# Autodesk Inventor assembly: 외곽프레임
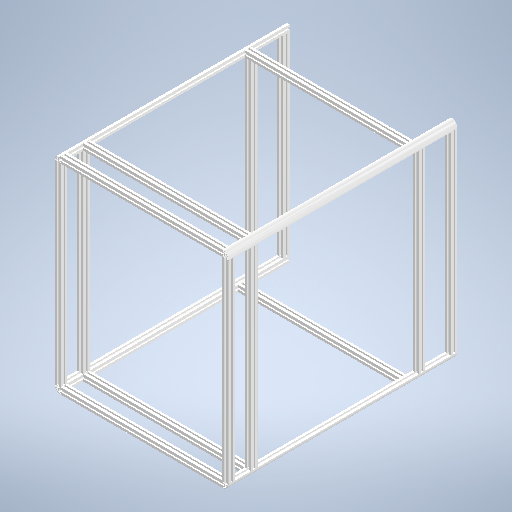
[picture p0: Inventor's stored thumbnail of the model, 512x512]
Saved by Autodesk Inventor 2025.4 (Build 294407000, 407)
## iProperties
Created: 2026-06-05
Part Number: 외곽프레임
Document SubType Name: Assembly
Designer: dalbi
Author: dalbi
## Documents named in this file (4)
- C:\Users\dalbi\OneDrive\바탕 화면\트리보 설계파일\최종 설계 파일(조립시 참고할 파일)\외곽프레임.iam
- C:\Users\dalbi\OneDrive\바탕 화면\트리보 설계파일\최종 설계 파일(조립시 참고할 파일)\AL_Profile_Round_20X20_710.ipt
- C:\Users\dalbi\OneDrive\바탕 화면\트리보 설계파일\최종 설계 파일(조립시 참고할 파일)\AL_Profile_20X20_600.ipt
- C:\Users\dalbi\OneDrive\바탕 화면\트리보 설계파일\최종 설계 파일(조립시 참고할 파일)\AL_Profile_20X20_500.ipt
## Components (18 placed, 3 different names)
1. AL_Profile_Round_20X20_710:1 — 플러쉬:1, 메이트:1, 각도:1, 메이트:2, 각도:2, 플러쉬:2, 플러쉬:7, 메이트:24, 플러쉬:24, 플러쉬:25, 메이트:25, 메이트:30, 플러쉬:34
2. AL_Profile_Round_20X20_710:2 — 플러쉬:1, 메이트:1, 각도:1, 플러쉬:4, 플러쉬:6, 플러쉬:7, 메이트:5, 플러쉬:10, 플러쉬:14, 메이트:10, 플러쉬:15, 플러쉬:26
3. AL_Profile_Round_20X20_710:3 — 각도:3, 메이트:3, 플러쉬:3, 플러쉬:4, 플러쉬:5, 플러쉬:6, 메이트:4, 플러쉬:8, 플러쉬:9, 플러쉬:16, 메이트:18, 플러쉬:23
4. AL_Profile_Round_20X20_710:4 — 메이트:2, 각도:2, 각도:3, 메이트:3, 플러쉬:2, 플러쉬:3, 플러쉬:5, 플러쉬:11, 메이트:6, 플러쉬:12, 플러쉬:13, 메이트:7, 플러쉬:17, 메이트:19, 플러쉬:18, 메이트:20, 플러쉬:19, 플러쉬:21, 메이트:26, 플러쉬:28, 메이트:27, 플러쉬:30
5. AL_Profile_20X20_600:1 — 메이트:4, 플러쉬:8, 플러쉬:9, 메이트:28
6. AL_Profile_20X20_600:2 — 플러쉬:11, 메이트:6, 플러쉬:12, 메이트:8
7. AL_Profile_20X20_600:3 — 메이트:17, 플러쉬:16, 메이트:18, 플러쉬:27
8. AL_Profile_20X20_600:4 — 메이트:5, 플러쉬:10, 메이트:28, 메이트:31
9. AL_Profile_20X20_600:5 — 플러쉬:14, 메이트:10, 플러쉬:15, 메이트:17
10. AL_Profile_20X20_600:6 — 플러쉬:13, 메이트:7, 메이트:8, 메이트:22, 플러쉬:35
11. AL_Profile_20X20_600:7 — 플러쉬:17, 메이트:19, 플러쉬:18, 메이트:21
12. AL_Profile_20X20_600:8 — 메이트:20, 플러쉬:19, 메이트:21, 플러쉬:29
13. AL_Profile_20X20_500:1 — 메이트:22, 플러쉬:21, 플러쉬:23
14. AL_Profile_20X20_500:3 — 메이트:26, 플러쉬:28, 플러쉬:29
15. AL_Profile_20X20_500:4 — 메이트:27, 플러쉬:30, 메이트:31
16. AL_Profile_20X20_500:5 — 메이트:24, 플러쉬:24, 플러쉬:25
17. AL_Profile_20X20_500:6 — 메이트:25, 플러쉬:26, 플러쉬:27
18. AL_Profile_20X20_500:8 — 메이트:30, 플러쉬:34, 플러쉬:35
## Relationships (55: Flush 30, Mate 22, Angle 3)
- 플러쉬:1 [Flush]: AL_Profile_Round_20X20_710:1 ↔ AL_Profile_Round_20X20_710:2
- 메이트:1 [Mate] (500 mm): AL_Profile_Round_20X20_710:1 ↔ AL_Profile_Round_20X20_710:2
- 각도:1 [Angle] (0 deg): AL_Profile_Round_20X20_710:1 ↔ AL_Profile_Round_20X20_710:2
- 메이트:2 [Mate] (600 mm): AL_Profile_Round_20X20_710:1 ↔ AL_Profile_Round_20X20_710:4
- 각도:2 [Angle] (0 deg): AL_Profile_Round_20X20_710:1 ↔ AL_Profile_Round_20X20_710:4
- 각도:3 [Angle] (0 deg): AL_Profile_Round_20X20_710:3 ↔ AL_Profile_Round_20X20_710:4
- 메이트:3 [Mate] (500 mm): AL_Profile_Round_20X20_710:3 ↔ AL_Profile_Round_20X20_710:4
- 플러쉬:2 [Flush]: AL_Profile_Round_20X20_710:1 ↔ AL_Profile_Round_20X20_710:4
- 플러쉬:3 [Flush]: AL_Profile_Round_20X20_710:3 ↔ AL_Profile_Round_20X20_710:4
- 플러쉬:4 [Flush]: AL_Profile_Round_20X20_710:2 ↔ AL_Profile_Round_20X20_710:3
- 플러쉬:5 [Flush]: AL_Profile_Round_20X20_710:3 ↔ AL_Profile_Round_20X20_710:4
- 플러쉬:6 [Flush]: AL_Profile_Round_20X20_710:2 ↔ AL_Profile_Round_20X20_710:3
- 플러쉬:7 [Flush]: AL_Profile_Round_20X20_710:1 ↔ AL_Profile_Round_20X20_710:2
- 메이트:4 [Mate]: AL_Profile_Round_20X20_710:3 ↔ AL_Profile_20X20_600:1
- 플러쉬:8 [Flush]: AL_Profile_Round_20X20_710:3 ↔ AL_Profile_20X20_600:1
- 플러쉬:9 [Flush]: AL_Profile_Round_20X20_710:3 ↔ AL_Profile_20X20_600:1
- 메이트:5 [Mate]: AL_Profile_Round_20X20_710:2 ↔ AL_Profile_20X20_600:4
- 플러쉬:10 [Flush]: AL_Profile_Round_20X20_710:2 ↔ AL_Profile_20X20_600:4
- 플러쉬:11 [Flush]: AL_Profile_Round_20X20_710:4 ↔ AL_Profile_20X20_600:2
- 메이트:6 [Mate]: AL_Profile_Round_20X20_710:4 ↔ AL_Profile_20X20_600:2
- 플러쉬:12 [Flush]: AL_Profile_Round_20X20_710:4 ↔ AL_Profile_20X20_600:2
- 플러쉬:13 [Flush]: AL_Profile_Round_20X20_710:4 ↔ AL_Profile_20X20_600:6
- 메이트:7 [Mate]: AL_Profile_Round_20X20_710:4 ↔ AL_Profile_20X20_600:6
- 메이트:8 [Mate] (80 mm): AL_Profile_20X20_600:2 ↔ AL_Profile_20X20_600:6
- 플러쉬:14 [Flush]: AL_Profile_Round_20X20_710:2 ↔ AL_Profile_20X20_600:5
- 메이트:10 [Mate]: AL_Profile_Round_20X20_710:2 ↔ AL_Profile_20X20_600:5
- 플러쉬:15 [Flush]: AL_Profile_Round_20X20_710:2 ↔ AL_Profile_20X20_600:5
- 메이트:17 [Mate] (50 mm): AL_Profile_20X20_600:3 ↔ AL_Profile_20X20_600:5
- 플러쉬:16 [Flush]: AL_Profile_Round_20X20_710:3 ↔ AL_Profile_20X20_600:3
- 메이트:18 [Mate]: AL_Profile_Round_20X20_710:3 ↔ AL_Profile_20X20_600:3
- 플러쉬:17 [Flush]: AL_Profile_Round_20X20_710:4 ↔ AL_Profile_20X20_600:7
- 메이트:19 [Mate]: AL_Profile_Round_20X20_710:4 ↔ AL_Profile_20X20_600:7
- 플러쉬:18 [Flush]: AL_Profile_Round_20X20_710:4 ↔ AL_Profile_20X20_600:7
- 메이트:20 [Mate]: AL_Profile_Round_20X20_710:4 ↔ AL_Profile_20X20_600:8
- 플러쉬:19 [Flush]: AL_Profile_Round_20X20_710:4 ↔ AL_Profile_20X20_600:8
- 메이트:21 [Mate] (50 mm): AL_Profile_20X20_600:7 ↔ AL_Profile_20X20_600:8
- 메이트:22 [Mate]: AL_Profile_20X20_600:6 ↔ AL_Profile_20X20_500:1
- 플러쉬:21 [Flush]: AL_Profile_Round_20X20_710:4 ↔ AL_Profile_20X20_500:1
- 플러쉬:23 [Flush]: AL_Profile_Round_20X20_710:3 ↔ AL_Profile_20X20_500:1
- 메이트:24 [Mate]: AL_Profile_Round_20X20_710:1 ↔ AL_Profile_20X20_500:5
- 플러쉬:24 [Flush]: AL_Profile_Round_20X20_710:1 ↔ AL_Profile_20X20_500:5
- 플러쉬:25 [Flush]: AL_Profile_Round_20X20_710:1 ↔ AL_Profile_20X20_500:5
- 메이트:25 [Mate]: AL_Profile_Round_20X20_710:1 ↔ AL_Profile_20X20_500:6
- 플러쉬:26 [Flush]: AL_Profile_Round_20X20_710:2 ↔ AL_Profile_20X20_500:6
- 플러쉬:27 [Flush]: AL_Profile_20X20_600:3 ↔ AL_Profile_20X20_500:6
- 메이트:26 [Mate]: AL_Profile_Round_20X20_710:4 ↔ AL_Profile_20X20_500:3
- 플러쉬:28 [Flush]: AL_Profile_Round_20X20_710:4 ↔ AL_Profile_20X20_500:3
- 플러쉬:29 [Flush]: AL_Profile_20X20_600:8 ↔ AL_Profile_20X20_500:3
- 메이트:27 [Mate]: AL_Profile_Round_20X20_710:4 ↔ AL_Profile_20X20_500:4
- 플러쉬:30 [Flush]: AL_Profile_Round_20X20_710:4 ↔ AL_Profile_20X20_500:4
- 메이트:28 [Mate] (80 mm): AL_Profile_20X20_600:1 ↔ AL_Profile_20X20_600:4
- 메이트:30 [Mate]: AL_Profile_Round_20X20_710:1 ↔ AL_Profile_20X20_500:8
- 플러쉬:34 [Flush]: AL_Profile_Round_20X20_710:1 ↔ AL_Profile_20X20_500:8
- 플러쉬:35 [Flush] (-20 mm): AL_Profile_20X20_600:6 ↔ AL_Profile_20X20_500:8
- 메이트:31 [Mate] (20 mm): AL_Profile_20X20_600:4 ↔ AL_Profile_20X20_500:4
